# Autodesk Inventor assembly: SAM2
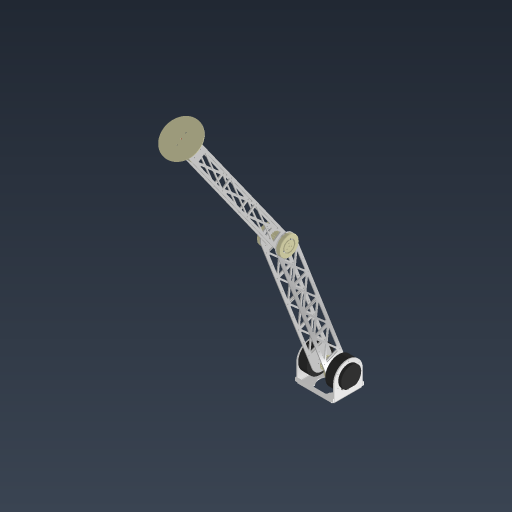
[picture p0: Inventor's stored thumbnail of the model, 512x512]
Saved by Autodesk Inventor 2024.1 (Build 281209000, 209)
## iProperties
Created: 2023-02-16
Part Number: SAM2
Document SubType Name: Assembly
Designer: dzw04
Author: dzw04
## Documents named in this file (15)
- C:\Users\dzw04\Saxion\Mechatronica Lectoraat LMECH LED - Database ARG\Component_Database\SAM2\01. CAD\01. 3D_Drawing\SAM2.iam
- C:\Users\dzw04\Saxion\Mechatronica Lectoraat LMECH LED - Database ARG\Component_Database\SAM2\01. CAD\01. 3D_Drawing\01. Parts\Motor_Mount.ipt
- C:\Users\dzw04\Saxion\Mechatronica Lectoraat LMECH LED - Database ARG\Component_Database\SAM2\01. CAD\01. 3D_Drawing\02. Sub_Assemblies\AK60-6.iam
- C:\Users\dzw04\Saxion\Mechatronica Lectoraat LMECH LED - Database ARG\Component_Database\SAM2\01. CAD\01. 3D_Drawing\01. Parts\Lower_Arm_Motor_Side.ipt
- C:\Users\dzw04\Saxion\Mechatronica Lectoraat LMECH LED - Database ARG\Component_Database\SAM2\01. CAD\01. 3D_Drawing\01. Parts\Lower_Arm_Bearing_Side.ipt
- C:\Users\dzw04\Saxion\Mechatronica Lectoraat LMECH LED - Database ARG\Component_Database\SAM2\01. CAD\01. 3D_Drawing\01. Parts\Bearing_Holder.ipt
- C:\Users\dzw04\Saxion\Mechatronica Lectoraat LMECH LED - Testomgeving van Dion\Component_Database\SAM2\01. Drawings\SAM2\Design Accelerator\Bearing1.iam
- C:\Users\dzw04\Saxion\Mechatronica Lectoraat LMECH LED - Database ARG\Component_Database\SAM2\01. CAD\01. 3D_Drawing\01. Parts\Shaft_Joint1.ipt
- C:\Users\dzw04\Saxion\Mechatronica Lectoraat LMECH LED - Database ARG\Component_Database\SAM2\01. CAD\01. 3D_Drawing\01. Parts\Pulley_Joint1.ipt
- C:\Users\dzw04\Saxion\Mechatronica Lectoraat LMECH LED - Database ARG\Component_Database\SAM2\01. CAD\01. 3D_Drawing\01. Parts\Top_Arm.ipt
- C:\Users\dzw04\Saxion\Mechatronica Lectoraat LMECH LED - Database ARG\Component_Database\SAM2\01. CAD\01. 3D_Drawing\01. Parts\Pulley_Joint2.ipt
- C:\Users\dzw04\Saxion\Mechatronica Lectoraat LMECH LED - Database ARG\Component_Database\SAM2\01. CAD\01. 3D_Drawing\01. Parts\Shaft1_Joint1.ipt
- C:\Users\dzw04\Saxion\Mechatronica Lectoraat LMECH LED - Database ARG\Component_Database\SAM2\01. CAD\01. 3D_Drawing\01. Parts\Shaft2_Joint2.ipt
- C:\Users\dzw04\Saxion\Mechatronica Lectoraat LMECH LED - Database ARG\Component_Database\SAM2\01. CAD\01. 3D_Drawing\01. Parts\Tool_Holder.ipt
- C:\Users\dzw04\Saxion\Mechatronica Lectoraat LMECH LED - Database ARG\Component_Database\SAM2\01. CAD\01. 3D_Drawing\02. Sub_Assemblies\End_Effector.iam
## Components (20 placed, 14 different names)
1. Motor_Mount:1 — Mate:1, Mate:2, Mate:3, Mate:4, Mate:5, Mate:6
2. AK60-6:1 [sub-assembly] — Mate:4, Mate:5, Mate:6, Mate:7, Mate:8, Mate:9
3. AK60-6:2 [sub-assembly] — Mate:1, Mate:2, Mate:3, Rigid:1
4. Lower_Arm_Motor_Side:1 — Mate:7, Mate:8, Mate:9, Mate:10, Mate:11, Mate:12, Mate:21, Mate:22, Mate:23, Rotational:1
5. Lower_Arm_Bearing_Side:1 — Mate:10, Mate:11, Mate:12, Mate:19, Mate:20, Mate:24, Mate:25, Mate:27
6. Bearing_Holder:1 — Mate:25, Mate:27
7. Bearing1:1 [sub-assembly]
8. Bearing_Holder:2 — Mate:21, Mate:23
9. Bearing1:2 [sub-assembly] — Mate:22
10. Bearing_Holder:3 — Mate:19, Mate:24
11. Bearing1:3 [sub-assembly] — Mate:20
12. Shaft_Joint1:1 — Mate:28, Mate:29, Mate:30, Rigid:1
13. Pulley_Joint1:1 — Mate:28, Mate:29, Mate:30
14. Top_Arm:1 — Mate:31, Mate:32, Mate:33, Mate:34, Mate:35, Mate:36, Mate:37, Mate:39, Flush:2
15. Top_Arm:2 — Mate:31, Mate:32, Mate:33, Rotational:1, Mate:38, Mate:43, Flush:1
16. Pulley_Joint2:1 — Mate:34, Mate:35, Mate:36
17. Shaft1_Joint1:2 — Mate:37, Mate:38, Mate:39, Mate:40, Mate:41, Mate:42
18. Shaft2_Joint2:1 — Mate:40, Mate:41, Mate:42
19. Tool_Holder:1 — Mate:43, Flush:1, Flush:2, Mate:44, Mate:45, Mate:46
20. End_Effector:1 [sub-assembly] — Mate:44, Mate:45, Mate:46
## Relationships (50: Mate 46, Flush 2, WeldJoint 1, RevoluteJoint 1)
- Mate:1: Motor_Mount:1 ↔ AK60-6:2
- Mate:2: Motor_Mount:1 ↔ AK60-6:2
- Mate:3: Motor_Mount:1 ↔ AK60-6:2
- Mate:4: Motor_Mount:1 ↔ AK60-6:1
- Mate:5: Motor_Mount:1 ↔ AK60-6:1
- Mate:6: Motor_Mount:1 ↔ AK60-6:1
- Mate:7: AK60-6:1 ↔ Lower_Arm_Motor_Side:1
- Mate:8: AK60-6:1 ↔ Lower_Arm_Motor_Side:1
- Mate:9: AK60-6:1 ↔ Lower_Arm_Motor_Side:1
- Mate:10 (40 mm): Lower_Arm_Motor_Side:1 ↔ Lower_Arm_Bearing_Side:1
- Mate:11: Lower_Arm_Motor_Side:1 ↔ Lower_Arm_Bearing_Side:1
- Mate:12: Lower_Arm_Motor_Side:1 ↔ Lower_Arm_Bearing_Side:1
- [Mate]: Bearing_Holder:1 ↔ Bearing1:1
- [Mate]: Bearing_Holder:1 ↔ Bearing1:1
- [Mate]: Bearing_Holder:2 ↔ Bearing1:2
- [Mate]: Bearing_Holder:2 ↔ Bearing1:2
- [Mate]: Bearing_Holder:3 ↔ Bearing1:3
- [Mate]: Bearing_Holder:3 ↔ Bearing1:3
- Mate:19: Lower_Arm_Bearing_Side:1 ↔ Bearing_Holder:3
- Mate:20: Lower_Arm_Bearing_Side:1 ↔ Bearing1:3
- Mate:21: Lower_Arm_Motor_Side:1 ↔ Bearing_Holder:2
- Mate:22: Lower_Arm_Motor_Side:1 ↔ Bearing1:2
- Mate:23: Lower_Arm_Motor_Side:1 ↔ Bearing_Holder:2
- Mate:24: Lower_Arm_Bearing_Side:1 ↔ Bearing_Holder:3
- Mate:25: Lower_Arm_Bearing_Side:1 ↔ Bearing_Holder:1
- [Mate]: Lower_Arm_Bearing_Side:1 ↔ Bearing1:1
- Mate:27: Lower_Arm_Bearing_Side:1 ↔ Bearing_Holder:1
- Mate:28: Shaft_Joint1:1 ↔ Pulley_Joint1:1
- Mate:29: Shaft_Joint1:1 ↔ Pulley_Joint1:1
- Mate:30: Shaft_Joint1:1 ↔ Pulley_Joint1:1
- Rigid:1 [WeldJoint]: AK60-6:2 ↔ Shaft_Joint1:1
- Mate:31 (20 mm): Top_Arm:1 ↔ Top_Arm:2
- Mate:32: Top_Arm:1 ↔ Top_Arm:2
- Mate:33: Top_Arm:1 ↔ Top_Arm:2
- Mate:34: Top_Arm:1 ↔ Pulley_Joint2:1
- Mate:35: Top_Arm:1 ↔ Pulley_Joint2:1
- Mate:36: Top_Arm:1 ↔ Pulley_Joint2:1
- Rotational:1 [RevoluteJoint] (7 mm): Lower_Arm_Motor_Side:1 ↔ Top_Arm:2
- Mate:37: Top_Arm:1 ↔ Shaft1_Joint1:2
- Mate:38: Top_Arm:2 ↔ Shaft1_Joint1:2
- Mate:39: Top_Arm:1 ↔ Shaft1_Joint1:2
- Mate:40: Shaft1_Joint1:2 ↔ Shaft2_Joint2:1
- Mate:41: Shaft1_Joint1:2 ↔ Shaft2_Joint2:1
- Mate:42: Shaft1_Joint1:2 ↔ Shaft2_Joint2:1
- Mate:43: Top_Arm:2 ↔ Tool_Holder:1
- Flush:1: Top_Arm:2 ↔ Tool_Holder:1
- Flush:2: Top_Arm:1 ↔ Tool_Holder:1
- Mate:44: Tool_Holder:1 ↔ End_Effector:1
- Mate:45: Tool_Holder:1 ↔ End_Effector:1
- Mate:46: Tool_Holder:1 ↔ End_Effector:1
## Named parameters: d14_d12 = 0 mm, d15_d13 = 0 mm, d16_d12 = 0 mm, d17_d13 = 0 mm
